# Autodesk Inventor assembly: 300145
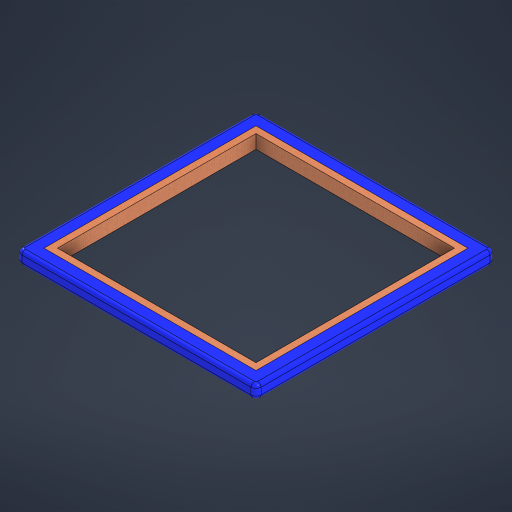
[picture p0: Inventor's stored thumbnail of the model, 512x512]
Saved by Autodesk Inventor 2023.1 (Build 271208000, 208)
## iProperties
Created: 2023-01-06
Part Number: 300145
Document SubType Name: Assembly
Designer: Byron Robotics
Mass: 11471.6 g
Surface Area: 11137.2 cm^2
Volume: 12423.3 cm^3
Density: 0.923389 g/cm^3
Author: Byron Robotics
## Documents named in this file (3)
- C:\$WorkingFolder\Projects\2022\Offseason\Swerve Drive\300145.iam
- C:\$WorkingFolder\Projects\2022\Offseason\Swerve Drive\200554.ipt
- C:\$WorkingFolder\Projects\2022\Offseason\Swerve Drive\200555.ipt
## Components (2 placed, 2 different names)
1. 200554:1 — Mate:1, Mate:2, Flush:1
2. 200555:1 — Mate:1, Mate:2, Flush:1
## Relationships (3: Mate 2, Flush 1)
- Mate:1: 200554:1 ↔ 200555:1
- Mate:2: 200554:1 ↔ 200555:1
- Flush:1: 200554:1 ↔ 200555:1
